# Autodesk Inventor assembly: frameAssembly
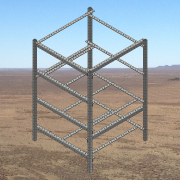
[picture p0: Inventor's stored thumbnail of the model, 180x180]
Saved by Autodesk Inventor 2014 SP1 (Build 180222100, 222)
## iProperties
Created: 2014-05-23
Part Number: frameAssembly
Document SubType Name: Assembly
Designer: Dave
Author: Dave
## Documents named in this file (4)
- C:\Users\Dave\Desktop\hera-cad\Node\frameAssembly.iam
- C:\Users\Dave\Desktop\hera-cad\Node\frame_uni_vert.ipt
- C:\Users\Dave\Desktop\hera-cad\Node\frame_angle_horiz.ipt
- C:\Users\Dave\Desktop\hera-cad\Node\frame_angle_horiz_short.ipt
## Components (22 placed, 3 different names)
1. frame_uni_vert:1 — Insert:4
2. frame_uni_vert:2
3. frame_uni_vert:3 — Insert:3, Insert:5
4. frame_uni_vert:4 — Insert:6
5. frame_angle_horiz:4 — Insert:3
6. frame_angle_horiz:5
7. frame_angle_horiz:3 — Insert:4
8. frame_angle_horiz:6
9. frame_angle_horiz:2 — Insert:5
10. frame_angle_horiz:7 — Mate:4
11. frame_angle_horiz:9
12. frame_angle_horiz:10
13. frame_angle_horiz:1 — Insert:6
14. frame_angle_horiz:8 — Mate:3
15. frame_angle_horiz:11
16. frame_angle_horiz:12 — Mate:1, Mate:2
17. frame_angle_horiz_short:1 — Mate:1, Mate:2
18. frame_angle_horiz_short:11
19. frame_angle_horiz_short:12
20. frame_angle_horiz_short:13
21. frame_angle_horiz_short:5 — Mate:3, Mate:4
22. frame_angle_horiz_short:14
## Component patterns: vertical (4 elements), horizon1 (2 elements), horiz2 (2 elements), horiz3 (4 elements), horiz4 (4 elements), pam (4 elements), (2 elements, first: frame_angle_horiz_short:5)
## Relationships (8: Insert 4, Mate 4)
- Insert:3: frame_uni_vert:3 ↔ frame_angle_horiz:4
- Insert:4: frame_uni_vert:1 ↔ frame_angle_horiz:3
- Insert:5: frame_uni_vert:3 ↔ frame_angle_horiz:2
- Insert:6: frame_uni_vert:4 ↔ frame_angle_horiz:1
- Mate:1: frame_angle_horiz:12 ↔ frame_angle_horiz_short:1
- Mate:2: frame_angle_horiz:12 ↔ frame_angle_horiz_short:1
- Mate:3: frame_angle_horiz:8 ↔ frame_angle_horiz_short:5
- Mate:4: frame_angle_horiz:7 ↔ frame_angle_horiz_short:5
